# Autodesk Inventor assembly: 204
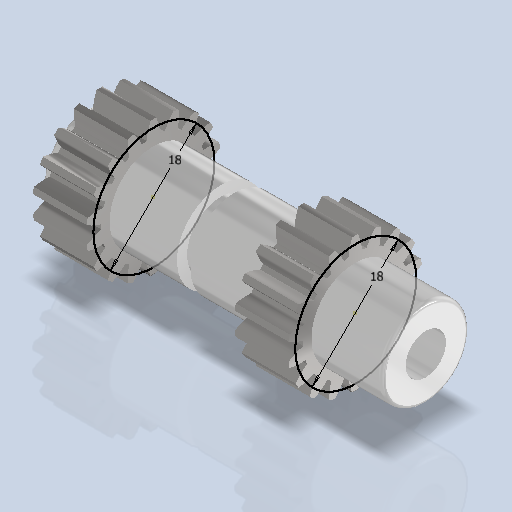
[picture p0: Inventor's stored thumbnail of the model, 512x512]
Saved by Autodesk Inventor 2024 (Build 280153000, 153)
## iProperties
Created: 2024-07-12
Part Number: 204
Document SubType Name: Assembly
Designer: ffogue
Author: ffogue
## Documents named in this file (3)
- C:\Users\ffogue\OneDrive - MuM - OM\Dokumente\Inventor\GearBox\204.iam
- C:\Users\ffogue\OneDrive - MuM - OM\Dokumente\Inventor\GearBox\204 Welle.ipt
- C:\Users\ffogue\OneDrive - MuM - OM\Dokumente\Inventor\GearBox\gear_204_18.iam
## Components (3 placed, 2 different names)
1. 204 Welle:1 — Einfügen:1, Einfügen:2
2. gear_204_18:1 [sub-assembly] — Einfügen:1
3. gear_204_18:2 [sub-assembly] — Einfügen:2
## Relationships (2: Insert 2)
- Einfügen:1 [Insert] (-18.5 mm): 204 Welle:1 ↔ gear_204_18:1
- Einfügen:2 [Insert] (-10 mm): 204 Welle:1 ↔ gear_204_18:2
